# Autodesk Inventor assembly: Arm 7DOF
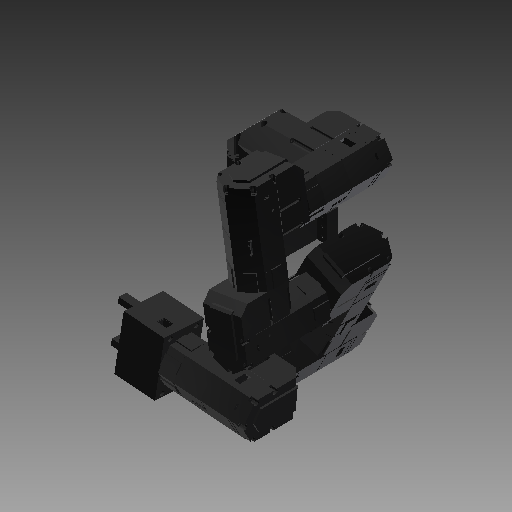
[picture p0: Inventor's stored thumbnail of the model, 512x512]
Saved by Autodesk Inventor 2017 (Build 210142000, 142)
## iProperties
Created: 2019-04-30
Part Number: Arm 7DOF
Document SubType Name: Assembly
Designer: Dell
Author: Dell
## Documents named in this file (6)
- C:\Users\Dell\Documents\GitHub\tr2\Arm\Arm 7DOF.iam
- C:\Users\Dell\Documents\GitHub\tr2\Gripper\Gripper.iam
- C:\Users\Dell\Documents\GitHub\tr2\Arm\TARM09b.ipt
- C:\Users\Dell\Documents\GitHub\tr2\Arm\TARM01b.ipt
- C:\Users\Dell\Documents\GitHub\tr2\Arm\TARM02b.ipt
- C:\Users\Dell\Documents\GitHub\tr2\Actuator 1.3\Actuator 1.3.iam
## Components (16 placed, 5 different names)
1. Gripper:1 [sub-assembly] — Mate:53, Mate:54
2. TARM09b:1 — Flush:1
3. TARM09b:2
4. TARM01b:1 — Mate:30, Mate:31, Mate:32
5. TARM02b:1
6. Actuator 1.3:1 [sub-assembly]
7. Actuator 1.3:2 [sub-assembly] — Mate:33, Mate:34
8. Actuator 1.3:3 [sub-assembly] — Mate:35, Mate:36, Mate:37
9. Actuator 1.3:4 [sub-assembly] — Mate:38, Mate:39
10. Actuator 1.3:5 [sub-assembly] — Mate:40, Mate:41, Mate:42, Mate:51, Mate:52
11. TARM09b:3 — Mate:33, Mate:34, Mate:35, Mate:36, Mate:37
12. TARM09b:4 — Mate:38, Mate:39, Mate:40, Mate:41, Mate:42
13. TARM09b:5 — Mate:51, Mate:52, Flush:1
14. Actuator 1.3:6 [sub-assembly]
15. Actuator 1.3:7 [sub-assembly] — Mate:53, Mate:54
16. TARM09b:6
## Relationships (43: Mate 42, Flush 1)
- [Mate]: TARM09b:1 ↔ TARM02b:1
- [Mate]: TARM09b:1 ↔ TARM02b:1
- [Mate]: TARM09b:1 ↔ TARM02b:1
- [Mate]: TARM01b:1 ↔ Actuator 1.3:1
- [Mate]: TARM01b:1 ↔ Actuator 1.3:1
- [Mate]: TARM01b:1 ↔ Actuator 1.3:1
- [Mate]: TARM02b:1 ↔ Actuator 1.3:1
- [Mate]: TARM02b:1 ↔ Actuator 1.3:1
- [Mate]: TARM09b:1 ↔ Actuator 1.3:2
- [Mate]: TARM09b:1 ↔ Actuator 1.3:2
- [Mate]: TARM09b:1 ↔ Actuator 1.3:2
- [Mate]: TARM09b:2 ↔ Actuator 1.3:3
- [Mate]: TARM09b:2 ↔ Actuator 1.3:3
- [Mate]: TARM09b:2 ↔ Actuator 1.3:4
- [Mate]: TARM09b:2 ↔ Actuator 1.3:4
- [Mate]: TARM09b:2 ↔ Actuator 1.3:4
- [Mate]: TARM01b:1 ↔ Actuator 1.3:1
- Mate:30: TARM01b:1
- Mate:31: TARM01b:1
- Mate:32: TARM01b:1
- Mate:33: Actuator 1.3:2 ↔ TARM09b:3
- Mate:34: Actuator 1.3:2 ↔ TARM09b:3
- Mate:35: Actuator 1.3:3 ↔ TARM09b:3
- Mate:36: Actuator 1.3:3 ↔ TARM09b:3
- Mate:37: Actuator 1.3:3 ↔ TARM09b:3
- Mate:38: Actuator 1.3:4 ↔ TARM09b:4
- Mate:39: Actuator 1.3:4 ↔ TARM09b:4
- Mate:40: Actuator 1.3:5 ↔ TARM09b:4
- Mate:41: Actuator 1.3:5 ↔ TARM09b:4
- Mate:42: Actuator 1.3:5 ↔ TARM09b:4
- [Mate]: TARM09b:5 ↔ Actuator 1.3:6
- [Mate]: TARM09b:5 ↔ Actuator 1.3:6
- [Mate]: TARM09b:5 ↔ Actuator 1.3:6
- [Mate]: Actuator 1.3:6 ↔ TARM09b:6
- [Mate]: Actuator 1.3:6 ↔ TARM09b:6
- [Mate]: Actuator 1.3:7 ↔ TARM09b:6
- [Mate]: Actuator 1.3:7 ↔ TARM09b:6
- [Mate]: Actuator 1.3:7 ↔ TARM09b:6
- Mate:51: Actuator 1.3:5 ↔ TARM09b:5
- Mate:52: Actuator 1.3:5 ↔ TARM09b:5
- Mate:53: Gripper:1 ↔ Actuator 1.3:7
- Mate:54: Gripper:1 ↔ Actuator 1.3:7
- Flush:1: TARM09b:1 ↔ TARM09b:5
## Named parameters: d42_d37 = 0 mm, d43_d38 = 0 mm, d44_d39 = 0 mm, d45_d40 = 0 mm, d46_d41 = 0 mm, d47_d359 = 0 mm, d48_d360 = 0 mm, d49_d361 = 0 mm
